# Autodesk Inventor assembly: SanladererBowdenExtruderMirrored
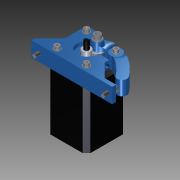
[picture p0: Inventor's stored thumbnail of the model, 180x180]
Saved by Autodesk Inventor 2015 SP1 (Build 190203100, 203)
## iProperties
Created: 2015-01-11
Part Number: SanladererBowdenExtruderMirrored
Document SubType Name: Assembly
Designer: Jack
Mass: 146.825 g
Surface Area: 300.593 cm^2
Volume: 138.026 cm^3
Density: 1.06375 g/cm^3
Author: Jack
Title: Sanlader Extruder Mirrored
## Documents named in this file (9)
- C:\Users\Jack\ownCloud\Projects\CrossBot\InventorModel\Extruder\SanladererBowdenExtruder\SanladererBowdenExtruderMirrored.iam
- C:\Users\Jack\ownCloud\Projects\CrossBot\InventorModel\Extruder\SanladererBowdenExtruder\SanladererBowdenBodyMirrored.ipt
- C:\Users\Jack\ownCloud\Projects\CrossBot\InventorModel\Extruder\SanladererBowdenExtruder\SanladererBowdenArmMirrored.ipt
- C:\Users\Jack\ownCloud\Projects\CrossBot\InventorModel\Hardware\Extruder\DriveGearMK8.ipt
- C:\Users\Jack\ownCloud\Projects\CrossBot\InventorModel\Hardware\Bearing\BearingRadialBall\BearingRadialBall624zz.ipt
- C:\Users\Jack\ownCloud\Projects\CrossBot\InventorModel\Hardware\BoltWashers\BoltWasher4\BoltWasher4x18.iam
- C:\Users\Jack\ownCloud\Projects\CrossBot\InventorModel\Hardware\BoltWashers\BoltWasher3\BoltWasher3x18.iam
- C:\Users\Jack\ownCloud\Projects\CrossBot\InventorModel\Hardware\BoltWashers\BoltWasher4\BoltWasher4x10.iam
- C:\Users\Jack\ownCloud\Projects\CrossBot\InventorModel\Electronics\Motors\StepperMotorNema17x60mm.ipt
## Components (12 placed, 8 different names)
1. SanladererBowdenBodyMirrored:1 — Mate:34, Mate:35, Mate:36, Mate:38, Mate:39, Mate:40, Mate:42, Mate:43, Mate:44, Mate:45, Mate:47
2. SanladererBowdenArmMirrored:1 — Mate:29, Mate:32, Mate:33, Mate:37, Mate:41
3. DriveGearMK8:1 — Flush:1
4. StepperMotorNema17x60mm:1 — Mate:47, Mate:48, Flush:1, Mate:49
5. BoltWasher3x18:1 [sub-assembly] — Mate:34, Mate:39, Mate:49
6. BoltWasher3x18:2 [sub-assembly] — Mate:35, Mate:38, Mate:48
7. BoltWasher3x18:3 [sub-assembly] — Mate:37, Mate:41
8. BoltWasher3x18:4 [sub-assembly] — Mate:36, Mate:40
9. BoltWasher4x10:1 [sub-assembly] — Mate:42, Mate:45
10. BoltWasher4x10:2 [sub-assembly] — Mate:43, Mate:44
11. BearingRadialBall624zz:1 — Mate:29, Mate:46
12. BoltWasher4x18:1 [sub-assembly] — Mate:32, Mate:33, Mate:46
## Relationships (20: Mate 19, Flush 1)
- Mate:29: SanladererBowdenArmMirrored:1 ↔ BearingRadialBall624zz:1
- Mate:32: SanladererBowdenArmMirrored:1 ↔ BoltWasher4x18:1
- Mate:33: SanladererBowdenArmMirrored:1 ↔ BoltWasher4x18:1
- Mate:34: SanladererBowdenBodyMirrored:1 ↔ BoltWasher3x18:1
- Mate:35: SanladererBowdenBodyMirrored:1 ↔ BoltWasher3x18:2
- Mate:36: SanladererBowdenBodyMirrored:1 ↔ BoltWasher3x18:4
- Mate:37: SanladererBowdenArmMirrored:1 ↔ BoltWasher3x18:3
- Mate:38: SanladererBowdenBodyMirrored:1 ↔ BoltWasher3x18:2
- Mate:39: SanladererBowdenBodyMirrored:1 ↔ BoltWasher3x18:1
- Mate:40: SanladererBowdenBodyMirrored:1 ↔ BoltWasher3x18:4
- Mate:41: SanladererBowdenArmMirrored:1 ↔ BoltWasher3x18:3
- Mate:42: SanladererBowdenBodyMirrored:1 ↔ BoltWasher4x10:1
- Mate:43: SanladererBowdenBodyMirrored:1 ↔ BoltWasher4x10:2
- Mate:44: SanladererBowdenBodyMirrored:1 ↔ BoltWasher4x10:2
- Mate:45: SanladererBowdenBodyMirrored:1 ↔ BoltWasher4x10:1
- Mate:46: BearingRadialBall624zz:1 ↔ BoltWasher4x18:1
- Mate:47: SanladererBowdenBodyMirrored:1 ↔ StepperMotorNema17x60mm:1
- Mate:48: StepperMotorNema17x60mm:1 ↔ BoltWasher3x18:2
- Flush:1 (-16 mm): DriveGearMK8:1 ↔ StepperMotorNema17x60mm:1
- Mate:49: StepperMotorNema17x60mm:1 ↔ BoltWasher3x18:1
